# Autodesk Inventor assembly: sort select and interface assembly
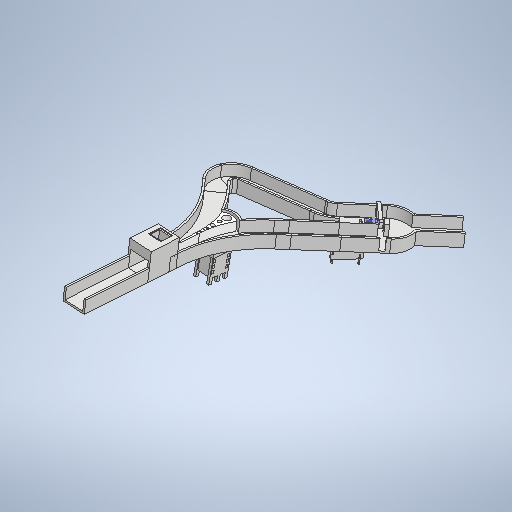
[picture p0: Inventor's stored thumbnail of the model, 512x512]
Saved by Autodesk Inventor 2025.3 (Build 293356000, 356)
## iProperties
Created: 2026-04-18
Part Number: sort select and interface assembly
Document SubType Name: Assembly
Designer: kamal
Author: kamal
## Documents named in this file (11)
- C:\Users\kamal\OneDrive\Desktop\Personal\semester 4\Basics of Mechatronics\Full Assembly\sort select and interface assembly.iam
- C:\Users\kamal\OneDrive\Desktop\Personal\semester 4\Basics of Mechatronics\Full Assembly\Sorting Full Mechanism.iam
- C:\Users\kamal\OneDrive\Desktop\Personal\semester 4\Basics of Mechatronics\Full Assembly\track 1832.ipt
- C:\Users\kamal\OneDrive\Desktop\Personal\semester 4\Basics of Mechatronics\Full Assembly\track z1906.ipt
- C:\Users\kamal\OneDrive\Desktop\Personal\semester 4\Basics of Mechatronics\Full Assembly\selection system 2.iam
- C:\Users\kamal\OneDrive\Desktop\Personal\semester 4\Basics of Mechatronics\Full Assembly\track z2029.ipt
- C:\Users\kamal\OneDrive\Desktop\Personal\semester 4\Basics of Mechatronics\Full Assembly\track z2053.ipt
- C:\Users\kamal\OneDrive\Desktop\Personal\semester 4\Basics of Mechatronics\Full Assembly\track z2059.ipt
- C:\Users\kamal\OneDrive\Desktop\Personal\semester 4\Basics of Mechatronics\Full Assembly\select end track.ipt
- C:\Users\kamal\OneDrive\Desktop\Personal\semester 4\Basics of Mechatronics\Full Assembly\holder 1.iam
- C:\Users\kamal\OneDrive\Desktop\Personal\semester 4\Basics of Mechatronics\Full Assembly\sort support V2.iam
## Components (11 placed, 10 different names)
1. Sorting Full Mechanism:1 [sub-assembly] — Mate:12, Mate:13, Mate:14, Mate:21, Mate:22, Mate:25, Mate:26, Mate:58, Mate:59, Mate:60
2. track 1832:1 — Mate:12, Mate:13, Mate:14
3. track z1906:1 — Mate:21, Mate:22, Mate:52, Mate:53
4. selection system 2:1 [sub-assembly] — Mate:27, Mate:28, Mate:41, Mate:42, Mate:54, Mate:55, Mate:56, Mate:57
5. track z2029:1 — Mate:25, Mate:26, Mate:27, Mate:28
6. track z1906:3 — Mate:35, Mate:36, Mate:52, Mate:53
7. track z2053:1 — Mate:35, Mate:36
8. track z2059:1 — Mate:54, Mate:55, Tangent:1
9. select end track:1 — Mate:41, Mate:42
10. holder 1:1 [sub-assembly] — Mate:56, Mate:57, Tangent:1
11. sort support V2:1 [sub-assembly] — Mate:58, Mate:59, Mate:60
## Relationships (23: Mate 22, Tangent 1)
- Mate:12: Sorting Full Mechanism:1 ↔ track 1832:1
- Mate:13: Sorting Full Mechanism:1 ↔ track 1832:1
- Mate:14: Sorting Full Mechanism:1 ↔ track 1832:1
- Mate:21: Sorting Full Mechanism:1 ↔ track z1906:1
- Mate:22: Sorting Full Mechanism:1 ↔ track z1906:1
- Mate:25: Sorting Full Mechanism:1 ↔ track z2029:1
- Mate:26: Sorting Full Mechanism:1 ↔ track z2029:1
- Mate:27: selection system 2:1 ↔ track z2029:1
- Mate:28: selection system 2:1 ↔ track z2029:1
- Mate:35: track z1906:3 ↔ track z2053:1
- Mate:36: track z1906:3 ↔ track z2053:1
- Mate:41: selection system 2:1 ↔ select end track:1
- Mate:42: selection system 2:1 ↔ select end track:1
- Mate:52: track z1906:1 ↔ track z1906:3
- Mate:53: track z1906:1 ↔ track z1906:3
- Mate:54: selection system 2:1 ↔ track z2059:1
- Mate:55: selection system 2:1 ↔ track z2059:1
- Mate:56: selection system 2:1 ↔ holder 1:1
- Mate:57: selection system 2:1 ↔ holder 1:1
- Tangent:1: track z2059:1 ↔ holder 1:1
- Mate:58: Sorting Full Mechanism:1 ↔ sort support V2:1
- Mate:59: Sorting Full Mechanism:1 ↔ sort support V2:1
- Mate:60: Sorting Full Mechanism:1 ↔ sort support V2:1
